# Autodesk Inventor assembly: assembly
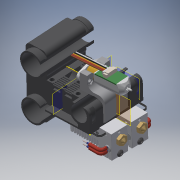
[picture p0: Inventor's stored thumbnail of the model, 180x180]
Saved by Autodesk Inventor 2019.4 (Build 234330000, 330)
## iProperties
Created: 2020-09-18
Part Number: assembly
Material: Generisch
Document SubType Name: Assembly
Designer: marc
Author: marc
## Documents named in this file (5)
- C:\Users\marc\Google Drive\Projekte\3D Drucker\brezzlicator\1. Printed Parts\3. Modified by marc\bltouch\assembly.iam
- C:\Users\marc\Google Drive\Projekte\3D Drucker\brezzlicator\1. Printed Parts\3. Modified by marc\x_carriage_aio_base 2.0.ipt
- C:\Users\marc\Google Drive\Projekte\3D Drucker\brezzlicator\1. Printed Parts\3. Modified by marc\bltouch\bltouch_mount_aio_base.ipt
- C:\Users\marc\Downloads\BLTouch-Smart V3.1.ipt
- C:\Users\marc\Google Drive\Projekte\3D Drucker\brezzlicator\1. Printed Parts\3. Modified by marc\titan_direct_drive_extruder\grabcad\Chimera+ Assembly MK1 v3.ipt
## Components (4 placed, 4 different names)
1. x_carriage_aio_base 2.0:1 — Drehbar:1, Drehbar:3
2. bltouch_mount_aio_base:1 — Drehbar:1, Drehbar:2
3. BLTouch-Smart V3.1:1 — Drehbar:2
4. Chimera+ Assembly MK1 v3:1 — Drehbar:3
## Relationships (3: RevoluteJoint 3)
- Drehbar:1 [RevoluteJoint]: x_carriage_aio_base 2.0:1 ↔ bltouch_mount_aio_base:1
- Drehbar:2 [RevoluteJoint]: bltouch_mount_aio_base:1 ↔ BLTouch-Smart V3.1:1
- Drehbar:3 [RevoluteJoint]: x_carriage_aio_base 2.0:1 ↔ Chimera+ Assembly MK1 v3:1
